# Autodesk Inventor assembly: Cart
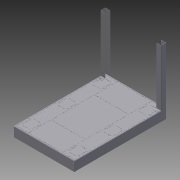
[picture p0: Inventor's stored thumbnail of the model, 180x180]
Saved by Autodesk Inventor 2012 (Build 160160000, 160)
## iProperties
Created: 2011-08-16
Part Number: Cart
Document SubType Name: Assembly
Designer: Ian Walters
Mass: 10168.7 g
Surface Area: 33651.2 cm^2
Volume: 3752.28 cm^3
Density: 2.71 g/cm^3
Author: Ian Walters
## Documents named in this file (21)
- E:\Preseason Projects\Cart Competition Cart\Cart.iam
- E:\Preseason Projects\Cart Competition Cart\Endrail.ipt
- E:\Preseason Projects\Cart Competition Cart\Inner Siderail.ipt
- E:\Preseason Projects\Cart Competition Cart\Outer Siderail.ipt
- E:\Preseason Projects\Cart Competition Cart\Top Sheet.ipt
- E:\Preseason Projects\Cart Competition Cart\Wheel Mount.ipt
- E:\Preseason Projects\Cart Competition Cart\Inner Endrail.ipt
- E:\Preseason Projects\Cart Competition Cart\Handle Support.ipt
- E:\Preseason Projects\Cart Competition Cart\Rear Endrail.ipt
- E:\Preseason Projects\Cart Competition Cart\Rear Wheel Mount.ipt
- E:\Preseason Projects\Cart Competition Cart\Rear Inner Endrail.ipt
- E:\Preseason Projects\Cart Competition Cart\Inner Siderail LHS.ipt
- E:\Preseason Projects\Cart Competition Cart\Outer Siderail LHS.ipt
- E:\Preseason Projects\Cart Competition Cart\Wheel Mount LHS.ipt
- E:\Preseason Projects\Cart Competition Cart\Handle Support LHS.ipt
- E:\Preseason Projects\Cart Competition Cart\Rear Wheel Mount LHS.ipt
- E:\Preseason Projects\Cart Competition Cart\IFI 114 - .1875  x .18.ipt
- E:\Preseason Projects\Cart Competition Cart\IFI 114 - .1875  x .27.ipt
- E:\Preseason Projects\Cart Competition Cart\Skeleton.ipt
- E:\Preseason Projects\Cart Competition Cart\IFI 114 - .1875  x .36.ipt
- IFI 114 - .1875  x .27.ipt
## Components (397 placed, 17 different names)
1. IFI 114 - .1875  x .27:131 — Insert:88
2. IFI 114 - .1875  x .27:132 — Insert:89
3. IFI 114 - .1875  x .27:133 — Insert:90
4. IFI 114 - .1875  x .27:134 — Insert:91
5. IFI 114 - .1875  x .27:135 — Insert:92
6. IFI 114 - .1875  x .27:136 — Insert:93
7. IFI 114 - .1875  x .27:137 — Insert:94
8. IFI 114 - .1875  x .27:138 — Insert:95
9. Handle Support:1 — Flush:19, Flush:20, Flush:21, Insert:8, Insert:9, Insert:15, Insert:16, Insert:88, Insert:89, Insert:94, Insert:95
10. Inner Endrail:1 — Flush:16, Flush:17, Flush:18
11. Wheel Mount:1 — Flush:13, Flush:14, Flush:15
12. Outer Siderail:1 — Flush:10, Flush:11, Flush:12
13. Inner Siderail:1 — Flush:7, Flush:8, Flush:9, Insert:20, Insert:21
14. Endrail:1 — Flush:4, Flush:5, Flush:6, Insert:2, Insert:3, Insert:4, Insert:5, Insert:6, Insert:7
15. Top Sheet:1 — Flush:1, Flush:2, Flush:3, Insert:1, Mate:1, Insert:22, Insert:23, Insert:24, Insert:25, Insert:26, Insert:27, Insert:28, Insert:29, Insert:30, Insert:31, Insert:32, Insert:33, Insert:34, Insert:35, Insert:36, Insert:37, Insert:38, Insert:39, Insert:40, Insert:41, Insert:42, Insert:43, Insert:44, Insert:45, Insert:46, Insert:47, Insert:48, Insert:49, Insert:50, Insert:51, Insert:52, Insert:53, Insert:54, Insert:55, Insert:56, Insert:57, Insert:58, Insert:59, Insert:60, Insert:61, Insert:62, Insert:63, Insert:64, Insert:65, Insert:66, Insert:67, Insert:68, Insert:69, Insert:70, Insert:71, Insert:72, Insert:73, Insert:74, Insert:75, Insert:76, Insert:77, Insert:78, Insert:79, Insert:80, Insert:81, Insert:82, Insert:83, Insert:84, Insert:85, Insert:86, Insert:87
16. Wheel Mount:2 — Insert:1, Mate:1
17. Rear Endrail:1 — Flush:22, Flush:23, Flush:24, Insert:10, Insert:13
18. Rear Wheel Mount:1 — Flush:25, Flush:26, Flush:27
19. Rear Inner Endrail:1 — Flush:28, Flush:29, Flush:30
20. Inner Siderail LHS:1 — Mate:2, Flush:31, Mate:3, Insert:18, Insert:19
21. Outer Siderail LHS:1 — Mate:4, Flush:32, Mate:5
22. Wheel Mount LHS:1 — Mate:6, Flush:33, Mate:7
23. Wheel Mount LHS:2
24. Handle Support LHS:1 — Mate:8, Flush:34, Mate:9, Insert:11, Insert:12, Insert:14, Insert:17, Insert:90, Insert:91, Insert:92, Insert:93
25. Rear Wheel Mount LHS:1 — Mate:10, Flush:35, Flush:36
26. IFI 114 - .1875  x .27:129 — Insert:66
27. IFI 114 - .1875  x .27:130 — Insert:67
28. IFI 114 - .1875  x .18:171 — Insert:50
29. IFI 114 - .1875  x .18:172 — Insert:51
30. IFI 114 - .1875  x .18:173 — Insert:52
31. IFI 114 - .1875  x .18:174 — Insert:53
32. IFI 114 - .1875  x .18:175 — Insert:54
33. IFI 114 - .1875  x .18:176 — Insert:55
34. IFI 114 - .1875  x .18:177 — Insert:56
35. IFI 114 - .1875  x .18:178 — Insert:57
36. IFI 114 - .1875  x .18:179 — Insert:58
37. IFI 114 - .1875  x .18:180 — Insert:59
38. IFI 114 - .1875  x .18:181 — Insert:60
39. IFI 114 - .1875  x .18:182 — Insert:61
40. IFI 114 - .1875  x .18:227 — Insert:72
41. IFI 114 - .1875  x .18:228 — Insert:73
42. IFI 114 - .1875  x .18:229 — Insert:74
43. IFI 114 - .1875  x .18:230 — Insert:75
44. IFI 114 - .1875  x .18:231 — Insert:76
45. IFI 114 - .1875  x .18:232 — Insert:77
46. IFI 114 - .1875  x .18:233 — Insert:78
47. IFI 114 - .1875  x .18:234 — Insert:79
48. IFI 114 - .1875  x .18:235 — Insert:80
49. IFI 114 - .1875  x .18:236 — Insert:81
50. IFI 114 - .1875  x .18:237 — Insert:82
51. IFI 114 - .1875  x .18:238 — Insert:83
52. IFI 114 - .1875  x .18:239 — Insert:84
53. IFI 114 - .1875  x .18:240 — Insert:85
54. IFI 114 - .1875  x .18:241 — Insert:86
55. IFI 114 - .1875  x .18:242 — Insert:87
56. IFI 114 - .1875  x .18:1 — Insert:2
57. IFI 114 - .1875  x .18:2 — Insert:3
58. IFI 114 - .1875  x .18:3 — Insert:4
59. IFI 114 - .1875  x .18:4 — Insert:5
60. IFI 114 - .1875  x .18:5 — Insert:6
61. IFI 114 - .1875  x .18:6 — Insert:7
62. IFI 114 - .1875  x .18:7 — Insert:8
63. IFI 114 - .1875  x .18:8 — Insert:9
64. IFI 114 - .1875  x .18:9 — Insert:10
65. IFI 114 - .1875  x .18:10 — Insert:11
66. IFI 114 - .1875  x .18:11 — Insert:12
67. IFI 114 - .1875  x .18:12 — Insert:13
68. IFI 114 - .1875  x .27:1 — Insert:14
69. IFI 114 - .1875  x .27:2 — Insert:15
70. IFI 114 - .1875  x .27:3 — Insert:16
71. IFI 114 - .1875  x .27:4 — Insert:17
72. IFI 114 - .1875  x .18:13 — Insert:18
73. IFI 114 - .1875  x .18:14 — Insert:19
74. IFI 114 - .1875  x .18:15 — Insert:20
75. IFI 114 - .1875  x .18:16 — Insert:21
76. IFI 114 - .1875  x .18:17
77. IFI 114 - .1875  x .18:18
78. IFI 114 - .1875  x .18:19
79. IFI 114 - .1875  x .18:20
80. IFI 114 - .1875  x .18:21
81. IFI 114 - .1875  x .18:22
82. IFI 114 - .1875  x .18:23
83. IFI 114 - .1875  x .18:24
84. IFI 114 - .1875  x .18:25
85. IFI 114 - .1875  x .18:26
86. IFI 114 - .1875  x .18:27
87. IFI 114 - .1875  x .18:28
88. IFI 114 - .1875  x .27:5
89. IFI 114 - .1875  x .27:6
90. IFI 114 - .1875  x .27:7
91. IFI 114 - .1875  x .27:8
92. IFI 114 - .1875  x .18:29
93. IFI 114 - .1875  x .18:30
94. IFI 114 - .1875  x .18:31
95. IFI 114 - .1875  x .18:32
96. IFI 114 - .1875  x .18:33
97. IFI 114 - .1875  x .18:34
98. IFI 114 - .1875  x .18:35
99. IFI 114 - .1875  x .18:36
100. IFI 114 - .1875  x .18:37
101. IFI 114 - .1875  x .18:38
102. IFI 114 - .1875  x .18:39
103. IFI 114 - .1875  x .18:40
104. IFI 114 - .1875  x .18:41
105. IFI 114 - .1875  x .18:42
106. IFI 114 - .1875  x .18:43
107. IFI 114 - .1875  x .18:44
108. IFI 114 - .1875  x .27:9
109. IFI 114 - .1875  x .27:10
110. IFI 114 - .1875  x .27:11
111. IFI 114 - .1875  x .27:12
112. IFI 114 - .1875  x .18:45
113. IFI 114 - .1875  x .18:46
114. IFI 114 - .1875  x .18:47
115. IFI 114 - .1875  x .18:48
116. IFI 114 - .1875  x .18:49
117. IFI 114 - .1875  x .18:50
118. IFI 114 - .1875  x .18:51
119. IFI 114 - .1875  x .18:52
120. IFI 114 - .1875  x .18:53
121. IFI 114 - .1875  x .18:54
122. IFI 114 - .1875  x .18:55
123. IFI 114 - .1875  x .18:56
124. IFI 114 - .1875  x .18:57
125. IFI 114 - .1875  x .18:58
126. IFI 114 - .1875  x .18:59
127. IFI 114 - .1875  x .18:60
128. IFI 114 - .1875  x .27:13
129. IFI 114 - .1875  x .27:14
130. IFI 114 - .1875  x .27:15
131. IFI 114 - .1875  x .27:16
132. IFI 114 - .1875  x .18:61
133. IFI 114 - .1875  x .18:62
134. IFI 114 - .1875  x .18:63
135. IFI 114 - .1875  x .18:64
136. IFI 114 - .1875  x .18:65
137. IFI 114 - .1875  x .18:66
138. IFI 114 - .1875  x .18:67
139. IFI 114 - .1875  x .18:68
140. IFI 114 - .1875  x .18:69
141. IFI 114 - .1875  x .18:70
142. IFI 114 - .1875  x .18:71
143. IFI 114 - .1875  x .18:72
144. IFI 114 - .1875  x .18:73
145. IFI 114 - .1875  x .18:74
146. IFI 114 - .1875  x .18:75
147. IFI 114 - .1875  x .18:76
148. IFI 114 - .1875  x .27:17
149. IFI 114 - .1875  x .27:18
150. IFI 114 - .1875  x .27:19
151. IFI 114 - .1875  x .27:20
152. IFI 114 - .1875  x .18:77
153. IFI 114 - .1875  x .18:78
154. IFI 114 - .1875  x .18:79
155. IFI 114 - .1875  x .18:80
156. IFI 114 - .1875  x .27:21 — Insert:22
157. IFI 114 - .1875  x .27:22 — Insert:23
158. IFI 114 - .1875  x .27:23 — Insert:24
159. IFI 114 - .1875  x .27:24 — Insert:25
160. IFI 114 - .1875  x .27:25 — Insert:26
161. IFI 114 - .1875  x .27:26 — Insert:29
162. IFI 114 - .1875  x .27:27 — Insert:27
163. IFI 114 - .1875  x .27:28 — Insert:28
164. IFI 114 - .1875  x .27:29
165. IFI 114 - .1875  x .27:30
166. IFI 114 - .1875  x .27:31
167. IFI 114 - .1875  x .27:32
168. IFI 114 - .1875  x .27:33
169. IFI 114 - .1875  x .27:34
170. IFI 114 - .1875  x .27:35
171. IFI 114 - .1875  x .27:36
172. IFI 114 - .1875  x .27:37
173. IFI 114 - .1875  x .27:38
174. IFI 114 - .1875  x .27:39
175. IFI 114 - .1875  x .27:40
176. IFI 114 - .1875  x .27:41
177. IFI 114 - .1875  x .27:42
178. IFI 114 - .1875  x .27:43
179. IFI 114 - .1875  x .27:44
180. IFI 114 - .1875  x .18:81 — Insert:30
181. IFI 114 - .1875  x .18:82 — Insert:31
182. IFI 114 - .1875  x .18:83 — Insert:32
183. IFI 114 - .1875  x .18:84 — Insert:33
184. IFI 114 - .1875  x .18:85 — Insert:34
185. IFI 114 - .1875  x .18:86 — Insert:35
186. IFI 114 - .1875  x .18:87 — Insert:36
187. IFI 114 - .1875  x .18:88 — Insert:37
188. IFI 114 - .1875  x .18:89 — Insert:38
189. IFI 114 - .1875  x .18:90 — Insert:39
190. IFI 114 - .1875  x .18:91
191. IFI 114 - .1875  x .18:92
192. IFI 114 - .1875  x .18:93
193. IFI 114 - .1875  x .18:94
194. IFI 114 - .1875  x .18:95
195. IFI 114 - .1875  x .18:96
196. IFI 114 - .1875  x .18:97
197. IFI 114 - .1875  x .18:98
198. IFI 114 - .1875  x .18:99
199. IFI 114 - .1875  x .18:100
200. IFI 114 - .1875  x .18:101
201. IFI 114 - .1875  x .18:102
202. IFI 114 - .1875  x .18:103
203. IFI 114 - .1875  x .18:104
204. IFI 114 - .1875  x .18:105
205. IFI 114 - .1875  x .18:106
206. IFI 114 - .1875  x .18:107
207. IFI 114 - .1875  x .18:108
208. IFI 114 - .1875  x .18:109
209. IFI 114 - .1875  x .18:110
210. IFI 114 - .1875  x .18:111
211. IFI 114 - .1875  x .18:112
212. IFI 114 - .1875  x .18:113
213. IFI 114 - .1875  x .18:114
214. IFI 114 - .1875  x .18:115
215. IFI 114 - .1875  x .18:116
216. IFI 114 - .1875  x .18:117
217. IFI 114 - .1875  x .18:118
218. IFI 114 - .1875  x .18:119
219. IFI 114 - .1875  x .18:120
220. IFI 114 - .1875  x .18:121 — Insert:40
221. IFI 114 - .1875  x .18:122 — Insert:41
222. IFI 114 - .1875  x .18:123 — Insert:42
223. IFI 114 - .1875  x .18:124 — Insert:43
224. IFI 114 - .1875  x .18:125 — Insert:44
225. IFI 114 - .1875  x .18:126 — Insert:45
226. IFI 114 - .1875  x .18:127 — Insert:46
227. IFI 114 - .1875  x .18:128 — Insert:47
228. IFI 114 - .1875  x .18:129 — Insert:48
229. IFI 114 - .1875  x .18:130 — Insert:49
230. IFI 114 - .1875  x .18:131
231. IFI 114 - .1875  x .18:132
232. IFI 114 - .1875  x .18:133
233. IFI 114 - .1875  x .18:134
234. IFI 114 - .1875  x .18:135
235. IFI 114 - .1875  x .18:136
236. IFI 114 - .1875  x .18:137
237. IFI 114 - .1875  x .18:138
238. IFI 114 - .1875  x .18:139
239. IFI 114 - .1875  x .18:140
240. IFI 114 - .1875  x .18:141
241. IFI 114 - .1875  x .18:142
242. IFI 114 - .1875  x .18:143
243. IFI 114 - .1875  x .18:144
244. IFI 114 - .1875  x .18:145
245. IFI 114 - .1875  x .18:146
246. IFI 114 - .1875  x .18:147
247. IFI 114 - .1875  x .18:148
248. IFI 114 - .1875  x .18:149
249. IFI 114 - .1875  x .18:150
250. IFI 114 - .1875  x .18:151
251. IFI 114 - .1875  x .18:152
252. IFI 114 - .1875  x .18:153
253. IFI 114 - .1875  x .18:154
254. IFI 114 - .1875  x .18:155
255. IFI 114 - .1875  x .18:156
256. IFI 114 - .1875  x .18:157
257. IFI 114 - .1875  x .18:158
258. IFI 114 - .1875  x .18:159
259. IFI 114 - .1875  x .18:160
260. IFI 114 - .1875  x .18:161
261. IFI 114 - .1875  x .18:162
262. IFI 114 - .1875  x .18:163
263. IFI 114 - .1875  x .18:164
264. IFI 114 - .1875  x .18:165
265. IFI 114 - .1875  x .18:166
266. IFI 114 - .1875  x .18:167
267. IFI 114 - .1875  x .18:168
268. IFI 114 - .1875  x .18:169
269. IFI 114 - .1875  x .18:170
270. IFI 114 - .1875  x .27:45 — Insert:62
271. IFI 114 - .1875  x .27:46 — Insert:63
272. IFI 114 - .1875  x .27:47 — Insert:64
273. IFI 114 - .1875  x .27:48 — Insert:65
274. IFI 114 - .1875  x .27:49
275. IFI 114 - .1875  x .27:50
276. IFI 114 - .1875  x .27:51
277. IFI 114 - .1875  x .27:52
278. IFI 114 - .1875  x .27:53
279. IFI 114 - .1875  x .27:54
280. IFI 114 - .1875  x .27:55
281. IFI 114 - .1875  x .27:56
282. IFI 114 - .1875  x .27:57
283. IFI 114 - .1875  x .27:58
284. IFI 114 - .1875  x .27:59
285. IFI 114 - .1875  x .27:60
286. IFI 114 - .1875  x .27:61
287. IFI 114 - .1875  x .27:62
288. IFI 114 - .1875  x .27:63
289. IFI 114 - .1875  x .27:64
290. IFI 114 - .1875  x .27:65
291. IFI 114 - .1875  x .27:66
292. IFI 114 - .1875  x .27:67
293. IFI 114 - .1875  x .27:68
294. IFI 114 - .1875  x .27:69
295. IFI 114 - .1875  x .27:70
296. IFI 114 - .1875  x .27:71
297. IFI 114 - .1875  x .27:72
298. IFI 114 - .1875  x .27:73
299. IFI 114 - .1875  x .27:74
300. IFI 114 - .1875  x .27:75
301. IFI 114 - .1875  x .27:76
302. IFI 114 - .1875  x .27:77
303. IFI 114 - .1875  x .27:78
304. IFI 114 - .1875  x .27:79
305. IFI 114 - .1875  x .27:80
306. IFI 114 - .1875  x .27:81
307. IFI 114 - .1875  x .27:82
308. IFI 114 - .1875  x .27:83
309. IFI 114 - .1875  x .27:84
310. IFI 114 - .1875  x .27:85
311. IFI 114 - .1875  x .27:86
312. IFI 114 - .1875  x .27:87
313. IFI 114 - .1875  x .27:88
314. IFI 114 - .1875  x .27:89
315. IFI 114 - .1875  x .27:90
316. IFI 114 - .1875  x .27:91
317. IFI 114 - .1875  x .27:92
318. IFI 114 - .1875  x .27:93
319. IFI 114 - .1875  x .27:94
320. IFI 114 - .1875  x .27:95
321. IFI 114 - .1875  x .27:96
322. IFI 114 - .1875  x .27:97
323. IFI 114 - .1875  x .27:98
324. IFI 114 - .1875  x .27:99
325. IFI 114 - .1875  x .27:100
326. IFI 114 - .1875  x .27:101
327. IFI 114 - .1875  x .27:102
328. IFI 114 - .1875  x .27:103
329. IFI 114 - .1875  x .27:104
330. IFI 114 - .1875  x .27:105
331. IFI 114 - .1875  x .27:106
332. IFI 114 - .1875  x .27:107
333. IFI 114 - .1875  x .27:108
334. IFI 114 - .1875  x .27:109
335. IFI 114 - .1875  x .27:110
336. IFI 114 - .1875  x .27:111
337. IFI 114 - .1875  x .27:112
338. IFI 114 - .1875  x .27:113
339. IFI 114 - .1875  x .27:114
340. IFI 114 - .1875  x .27:115
341. IFI 114 - .1875  x .27:116
342. IFI 114 - .1875  x .27:117
343. IFI 114 - .1875  x .27:118
344. IFI 114 - .1875  x .27:119
345. IFI 114 - .1875  x .27:120
346. IFI 114 - .1875  x .27:121
347. IFI 114 - .1875  x .27:122
348. IFI 114 - .1875  x .27:123
349. IFI 114 - .1875  x .27:124
350. IFI 114 - .1875  x .27:125
351. IFI 114 - .1875  x .27:126
352. IFI 114 - .1875  x .27:127
353. IFI 114 - .1875  x .27:128
354. IFI 114 - .1875  x .18:183 — Insert:68
355. IFI 114 - .1875  x .18:184 — Insert:69
356. IFI 114 - .1875  x .18:185 — Insert:70
357. IFI 114 - .1875  x .18:186 — Insert:71
358. IFI 114 - .1875  x .18:187
359. IFI 114 - .1875  x .18:188
360. IFI 114 - .1875  x .18:189
361. IFI 114 - .1875  x .18:190
362. IFI 114 - .1875  x .18:191
363. IFI 114 - .1875  x .18:192
364. IFI 114 - .1875  x .18:193
365. IFI 114 - .1875  x .18:194
366. IFI 114 - .1875  x .18:195
367. IFI 114 - .1875  x .18:196
368. IFI 114 - .1875  x .18:197
369. IFI 114 - .1875  x .18:198
370. IFI 114 - .1875  x .18:199
371. IFI 114 - .1875  x .18:200
372. IFI 114 - .1875  x .18:201
373. IFI 114 - .1875  x .18:202
374. IFI 114 - .1875  x .18:203
375. IFI 114 - .1875  x .18:204
376. IFI 114 - .1875  x .18:205
377. IFI 114 - .1875  x .18:206
378. IFI 114 - .1875  x .18:207
379. IFI 114 - .1875  x .18:208
380. IFI 114 - .1875  x .18:209
381. IFI 114 - .1875  x .18:210
382. IFI 114 - .1875  x .18:211
383. IFI 114 - .1875  x .18:212
384. IFI 114 - .1875  x .18:213
385. IFI 114 - .1875  x .18:214
386. IFI 114 - .1875  x .18:215
387. IFI 114 - .1875  x .18:216
388. IFI 114 - .1875  x .18:217
389. IFI 114 - .1875  x .18:218
390. IFI 114 - .1875  x .18:219
391. IFI 114 - .1875  x .18:220
392. IFI 114 - .1875  x .18:221
393. IFI 114 - .1875  x .18:222
394. IFI 114 - .1875  x .18:223
395. IFI 114 - .1875  x .18:224
396. IFI 114 - .1875  x .18:225
397. IFI 114 - .1875  x .18:226
## Component patterns: Side Rivets (5 elements), Top End Rivets (3 elements), Wheel Mount Rivets 1 (4 elements), Wheel Mount Rivets 2 (5 elements), Lengthwise Rivets (21 elements), (11 elements, first: IFI 114 - .1875  x .18:183 + IFI 114 - .1875  x .18:184 + IFI 114 - .1875  x .18:185 + IFI 114 - .1875  x .18:186)
## Relationships (141: Insert 95, Flush 36, Mate 10)
- Flush:1: Top Sheet:1
- Flush:2: Top Sheet:1
- Flush:3: Top Sheet:1
- Flush:4: Endrail:1
- Flush:5: Endrail:1
- Flush:6: Endrail:1
- Flush:7: Inner Siderail:1
- Flush:8: Inner Siderail:1
- Flush:9: Inner Siderail:1
- Flush:10: Outer Siderail:1
- Flush:11: Outer Siderail:1
- Flush:12: Outer Siderail:1
- Flush:13: Wheel Mount:1
- Flush:14: Wheel Mount:1
- Flush:15: Wheel Mount:1
- Flush:16: Inner Endrail:1
- Flush:17: Inner Endrail:1
- Flush:18: Inner Endrail:1
- Insert:1: Top Sheet:1 ↔ Wheel Mount:2
- Mate:1: Top Sheet:1 ↔ Wheel Mount:2
- Flush:19: Handle Support:1
- Flush:20: Handle Support:1
- Flush:21: Handle Support:1
- Flush:22: Rear Endrail:1
- Flush:23: Rear Endrail:1
- Flush:24: Rear Endrail:1
- Flush:25: Rear Wheel Mount:1
- Flush:26: Rear Wheel Mount:1
- Flush:27: Rear Wheel Mount:1
- Flush:28: Rear Inner Endrail:1
- Flush:29: Rear Inner Endrail:1
- Flush:30: Rear Inner Endrail:1
- Mate:2: Inner Siderail LHS:1
- Flush:31: Inner Siderail LHS:1
- Mate:3: Inner Siderail LHS:1
- Mate:4: Outer Siderail LHS:1
- Flush:32: Outer Siderail LHS:1
- Mate:5: Outer Siderail LHS:1
- Mate:6: Wheel Mount LHS:1
- Flush:33: Wheel Mount LHS:1
- Mate:7: Wheel Mount LHS:1
- Mate:8: Handle Support LHS:1
- Flush:34: Handle Support LHS:1
- Mate:9: Handle Support LHS:1
- Mate:10: Rear Wheel Mount LHS:1
- Flush:35: Rear Wheel Mount LHS:1
- Flush:36: Rear Wheel Mount LHS:1
- Insert:2: Endrail:1 ↔ IFI 114 - .1875  x .18:1
- Insert:3: Endrail:1 ↔ IFI 114 - .1875  x .18:2
- Insert:4: Endrail:1 ↔ IFI 114 - .1875  x .18:3
- Insert:5: Endrail:1 ↔ IFI 114 - .1875  x .18:4
- Insert:6: Endrail:1 ↔ IFI 114 - .1875  x .18:5
- Insert:7: Endrail:1 ↔ IFI 114 - .1875  x .18:6
- Insert:8: Handle Support:1 ↔ IFI 114 - .1875  x .18:7
- Insert:9: Handle Support:1 ↔ IFI 114 - .1875  x .18:8
- Insert:10: Rear Endrail:1 ↔ IFI 114 - .1875  x .18:9
- Insert:11: Handle Support LHS:1 ↔ IFI 114 - .1875  x .18:10
- Insert:12: Handle Support LHS:1 ↔ IFI 114 - .1875  x .18:11
- Insert:13: Rear Endrail:1 ↔ IFI 114 - .1875  x .18:12
- Insert:14: Handle Support LHS:1 ↔ IFI 114 - .1875  x .27:1
- Insert:15: Handle Support:1 ↔ IFI 114 - .1875  x .27:2
- Insert:16: Handle Support:1 ↔ IFI 114 - .1875  x .27:3
- Insert:17: Handle Support LHS:1 ↔ IFI 114 - .1875  x .27:4
- Insert:18: Inner Siderail LHS:1 ↔ IFI 114 - .1875  x .18:13
- Insert:19: Inner Siderail LHS:1 ↔ IFI 114 - .1875  x .18:14
- Insert:20: Inner Siderail:1 ↔ IFI 114 - .1875  x .18:15
- Insert:21: Inner Siderail:1 ↔ IFI 114 - .1875  x .18:16
- Insert:22: Top Sheet:1 ↔ IFI 114 - .1875  x .27:21
- Insert:23: Top Sheet:1 ↔ IFI 114 - .1875  x .27:22
- Insert:24: Top Sheet:1 ↔ IFI 114 - .1875  x .27:23
- Insert:25: Top Sheet:1 ↔ IFI 114 - .1875  x .27:24
- Insert:26: Top Sheet:1 ↔ IFI 114 - .1875  x .27:25
- Insert:27: Top Sheet:1 ↔ IFI 114 - .1875  x .27:27
- Insert:28: Top Sheet:1 ↔ IFI 114 - .1875  x .27:28
- Insert:29: Top Sheet:1 ↔ IFI 114 - .1875  x .27:26
- Insert:30: Top Sheet:1 ↔ IFI 114 - .1875  x .18:81
- Insert:31: Top Sheet:1 ↔ IFI 114 - .1875  x .18:82
- Insert:32: Top Sheet:1 ↔ IFI 114 - .1875  x .18:83
- Insert:33: Top Sheet:1 ↔ IFI 114 - .1875  x .18:84
- Insert:34: Top Sheet:1 ↔ IFI 114 - .1875  x .18:85
- Insert:35: Top Sheet:1 ↔ IFI 114 - .1875  x .18:86
- Insert:36: Top Sheet:1 ↔ IFI 114 - .1875  x .18:87
- Insert:37: Top Sheet:1 ↔ IFI 114 - .1875  x .18:88
- Insert:38: Top Sheet:1 ↔ IFI 114 - .1875  x .18:89
- Insert:39: Top Sheet:1 ↔ IFI 114 - .1875  x .18:90
- Insert:40: Top Sheet:1 ↔ IFI 114 - .1875  x .18:121
- Insert:41: Top Sheet:1 ↔ IFI 114 - .1875  x .18:122
- Insert:42: Top Sheet:1 ↔ IFI 114 - .1875  x .18:123
- Insert:43: Top Sheet:1 ↔ IFI 114 - .1875  x .18:124
- Insert:44: Top Sheet:1 ↔ IFI 114 - .1875  x .18:125
- Insert:45: Top Sheet:1 ↔ IFI 114 - .1875  x .18:126
- Insert:46: Top Sheet:1 ↔ IFI 114 - .1875  x .18:127
- Insert:47: Top Sheet:1 ↔ IFI 114 - .1875  x .18:128
- Insert:48: Top Sheet:1 ↔ IFI 114 - .1875  x .18:129
- Insert:49: Top Sheet:1 ↔ IFI 114 - .1875  x .18:130
- Insert:50: Top Sheet:1 ↔ IFI 114 - .1875  x .18:171
- Insert:51: Top Sheet:1 ↔ IFI 114 - .1875  x .18:172
- Insert:52: Top Sheet:1 ↔ IFI 114 - .1875  x .18:173
- Insert:53: Top Sheet:1 ↔ IFI 114 - .1875  x .18:174
- Insert:54: Top Sheet:1 ↔ IFI 114 - .1875  x .18:175
- Insert:55: Top Sheet:1 ↔ IFI 114 - .1875  x .18:176
- Insert:56: Top Sheet:1 ↔ IFI 114 - .1875  x .18:177
- Insert:57: Top Sheet:1 ↔ IFI 114 - .1875  x .18:178
- Insert:58: Top Sheet:1 ↔ IFI 114 - .1875  x .18:179
- Insert:59: Top Sheet:1 ↔ IFI 114 - .1875  x .18:180
- Insert:60: Top Sheet:1 ↔ IFI 114 - .1875  x .18:181
- Insert:61: Top Sheet:1 ↔ IFI 114 - .1875  x .18:182
- Insert:62: Top Sheet:1 ↔ IFI 114 - .1875  x .27:45
- Insert:63: Top Sheet:1 ↔ IFI 114 - .1875  x .27:46
- Insert:64: Top Sheet:1 ↔ IFI 114 - .1875  x .27:47
- Insert:65: Top Sheet:1 ↔ IFI 114 - .1875  x .27:48
- Insert:66: Top Sheet:1 ↔ IFI 114 - .1875  x .27:129
- Insert:67: Top Sheet:1 ↔ IFI 114 - .1875  x .27:130
- Insert:68: Top Sheet:1 ↔ IFI 114 - .1875  x .18:183
- Insert:69: Top Sheet:1 ↔ IFI 114 - .1875  x .18:184
- Insert:70: Top Sheet:1 ↔ IFI 114 - .1875  x .18:185
- Insert:71: Top Sheet:1 ↔ IFI 114 - .1875  x .18:186
- Insert:72: Top Sheet:1 ↔ IFI 114 - .1875  x .18:227
- Insert:73: Top Sheet:1 ↔ IFI 114 - .1875  x .18:228
- Insert:74: Top Sheet:1 ↔ IFI 114 - .1875  x .18:229
- Insert:75: Top Sheet:1 ↔ IFI 114 - .1875  x .18:230
- Insert:76: Top Sheet:1 ↔ IFI 114 - .1875  x .18:231
- Insert:77: Top Sheet:1 ↔ IFI 114 - .1875  x .18:232
- Insert:78: Top Sheet:1 ↔ IFI 114 - .1875  x .18:233
- Insert:79: Top Sheet:1 ↔ IFI 114 - .1875  x .18:234
- Insert:80: Top Sheet:1 ↔ IFI 114 - .1875  x .18:235
- Insert:81: Top Sheet:1 ↔ IFI 114 - .1875  x .18:236
- Insert:82: Top Sheet:1 ↔ IFI 114 - .1875  x .18:237
- Insert:83: Top Sheet:1 ↔ IFI 114 - .1875  x .18:238
- Insert:84: Top Sheet:1 ↔ IFI 114 - .1875  x .18:239
- Insert:85: Top Sheet:1 ↔ IFI 114 - .1875  x .18:240
- Insert:86: Top Sheet:1 ↔ IFI 114 - .1875  x .18:241
- Insert:87: Top Sheet:1 ↔ IFI 114 - .1875  x .18:242
- Insert:88: IFI 114 - .1875  x .27:131 ↔ Handle Support:1
- Insert:89: IFI 114 - .1875  x .27:132 ↔ Handle Support:1
- Insert:90: IFI 114 - .1875  x .27:133 ↔ Handle Support LHS:1
- Insert:91: IFI 114 - .1875  x .27:134 ↔ Handle Support LHS:1
- Insert:92: IFI 114 - .1875  x .27:135 ↔ Handle Support LHS:1
- Insert:93: IFI 114 - .1875  x .27:136 ↔ Handle Support LHS:1
- Insert:94: IFI 114 - .1875  x .27:137 ↔ Handle Support:1
- Insert:95: IFI 114 - .1875  x .27:138 ↔ Handle Support:1
## Named parameters: rivetSpacing = 12.7 mm
